# Autodesk Inventor assembly: bane bots wheel 3in
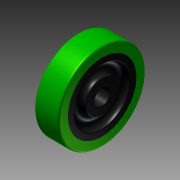
[picture p0: Inventor's stored thumbnail of the model, 180x180]
Saved by Autodesk Inventor 2012 (Build 160160000, 160)
## iProperties
Created: 2013-07-13
Part Number: bane bots wheel 3in
Document SubType Name: Assembly
Designer: Bryce
Author: Bryce
## Documents named in this file (3)
- C:\Users\Bryce\Dropbox\Inventor Design Project Files\Independent Swerves\Inventor 2012\bane bots wheel 3in.iam
- C:\Users\Bryce\Dropbox\Inventor Design Project Files\Independent Swerves\Inventor 2012\bane bots wheel hub 3 in.ipt
- C:\Users\Bryce\Dropbox\Inventor Design Project Files\Independent Swerves\Inventor 2012\bane bots wheel tread 3in.ipt
## Components (2 placed, 2 different names)
1. bane bots wheel hub 3 in:1 — Mate:1, Flush:1
2. bane bots wheel tread 3in:1 — Mate:1, Flush:1
## Relationships (2: Mate 1, Flush 1)
- Mate:1: bane bots wheel hub 3 in:1 ↔ bane bots wheel tread 3in:1
- Flush:1: bane bots wheel hub 3 in:1 ↔ bane bots wheel tread 3in:1
